# Autodesk Inventor assembly: AssemblyV1
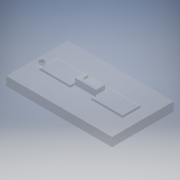
[picture p0: Inventor's stored thumbnail of the model, 180x180]
Saved by Autodesk Inventor 2017 (Build 210142000, 142)
## iProperties
Created: 2017-12-29
Part Number: AssemblyV1
Document SubType Name: Assembly
Designer: Tripl_000
Author: Tripl_000
## Documents named in this file (4)
- C:\Users\Tripl_000\Desktop\Spira\3D Models\2017\Optical Density Sensor Enclosure\Enclosure\Design 4\AssemblyV1.iam
- C:\Users\Tripl_000\Desktop\Spira\3D Models\2017\Optical Density Sensor Enclosure\Enclosure\Design 4\ODS_Enclosure_Bottom_V1D4.ipt
- C:\Users\Tripl_000\Desktop\Spira\3D Models\2017\Optical Density Sensor Enclosure\Enclosure\Design 4\ODS_Enclosure_Mid_V1D4.ipt
- C:\Users\Tripl_000\Desktop\Spira\3D Models\2017\Optical Density Sensor Enclosure\Enclosure\Design 4\ODS_Enclosure_Top_V1D4.ipt
## Components (3 placed, 3 different names)
1. ODS_Enclosure_Bottom_V1D4:1 — Mate:1, Mate:2
2. ODS_Enclosure_Mid_V1D4:1 — Mate:1, Mate:2, Mate:3, Mate:4
3. ODS_Enclosure_Top_V1D4:1 — Mate:3, Mate:4
## Relationships (4: Mate 4)
- Mate:1: ODS_Enclosure_Bottom_V1D4:1 ↔ ODS_Enclosure_Mid_V1D4:1
- Mate:2: ODS_Enclosure_Bottom_V1D4:1 ↔ ODS_Enclosure_Mid_V1D4:1
- Mate:3: ODS_Enclosure_Mid_V1D4:1 ↔ ODS_Enclosure_Top_V1D4:1
- Mate:4: ODS_Enclosure_Mid_V1D4:1 ↔ ODS_Enclosure_Top_V1D4:1
